# Autodesk Inventor assembly: ASY MSC 080 roсket
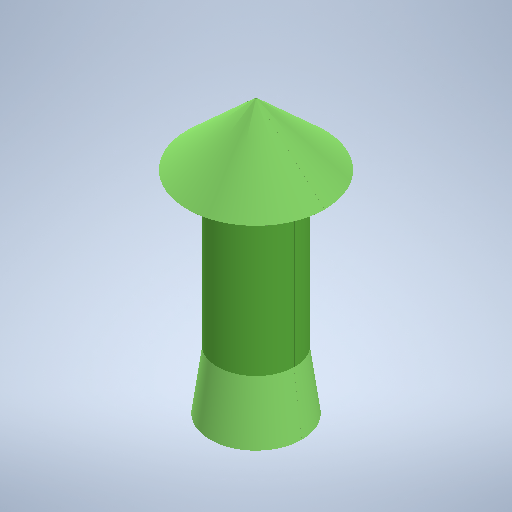
[picture p0: Inventor's stored thumbnail of the model, 512x512]
Saved by Autodesk Inventor 2025 (Build 290162010, 162A)
## iProperties
Created: 2024-05-19
Part Number: ASY MSC 080 roсket
Document SubType Name: Assembly
Designer: admin
Stock Number: МОО 080 диффузор отбойник
Author: admin
## Documents named in this file (5)
- C:\Users\user\YandexDisk\домашниий пк\Inventor\Manturovo\Manturovo_Se-clar\ASY MSC 080 roсket.iam
- C:\Users\user\YandexDisk\домашниий пк\Inventor\Manturovo\Manturovo_Se-clar\MSC DIM 084 roсket sketch.ipt
- C:\Users\user\YandexDisk\домашниий пк\Inventor\Manturovo\Manturovo_Se-clar\ракета\MSC 081 roсket tail.ipt
- C:\Users\user\YandexDisk\домашниий пк\Inventor\Manturovo\Manturovo_Se-clar\ракета\MSC 082 roсket body.ipt
- C:\Users\user\YandexDisk\домашниий пк\Inventor\Manturovo\Manturovo_Se-clar\ракета\MSC 083 roсket nose.ipt
## Components (4 placed, 4 different names)
1. MSC DIM 084 roсket sketch.ipt:1
2. MSC 081 roсket tail.ipt:1 — Rigid:1, Mate:2
3. MSC 082 roсket body.ipt:1 — Rigid:1, Rigid:2
4. MSC 083 roсket nose.ipt:1 — Rigid:2
## Relationships (3: WeldJoint 2, Mate 1)
- Rigid:1 [WeldJoint]: MSC 081 roсket tail.ipt:1 ↔ MSC 082 roсket body.ipt:1
- Rigid:2 [WeldJoint] (10 mm): MSC 082 roсket body.ipt:1 ↔ MSC 083 roсket nose.ipt:1
- Mate:2: MSC 081 roсket tail.ipt:1
